# Autodesk Inventor assembly: servo_holder-asm
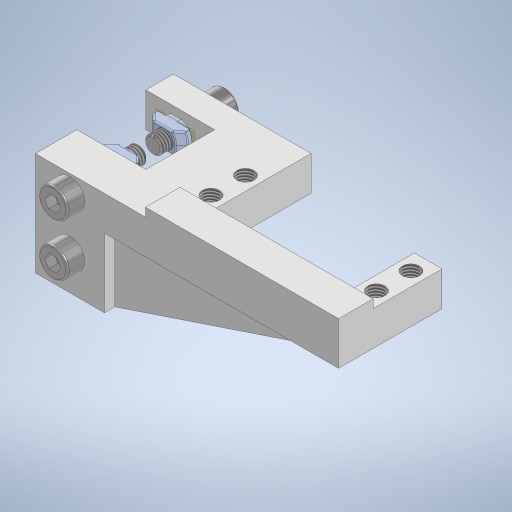
[picture p0: Inventor's stored thumbnail of the model, 512x512]
Saved by Autodesk Inventor 2024 (Build 280153000, 153)
## iProperties
Created: 2025-12-27
Part Number: servo_holder-asm
Document SubType Name: Assembly
Designer: schar
Author: schar
## Documents named in this file (5)
- C:\Users\schar\Desktop\projectBlueprint\AMSTS\hardware\servo_holder-asm.iam
- C:\Users\schar\Desktop\projectBlueprint\AMSTS\hardware\servo_holder.ipt
- C:\Users\schar\Desktop\projectBlueprint\AMSTS\hardware\tnut_m5_2020.ipt
- C:\Users\schar\Documents\Inventor\Content Center Files\R2024\en-US\ISO 4762(1)\DIN EN ISO 4762 - M5 x 20.ipt
- C:\Users\schar\Documents\Inventor\Content Center Files\R2024\en-US\ISO 4762(1)\DIN EN ISO 4762 - M5 x 16.ipt
## Components (7 placed, 4 different names)
1. servo_holder:1 — Rigid:3, Rigid:1, Rigid:2, Mate:1, Mate:2, Mate:3
2. tnut_m5_2020:1 — Rigid:2, Mate:4
3. tnut_m5_2020:2 — Rigid:1, Mate:6
4. tnut_m5_2020:3 — Rigid:3, Mate:5
5. DIN EN ISO 4762 M5 x 20:1 — Mate:1, Mate:6
6. DIN EN ISO 4762 M5 x 20:2 — Mate:2, Mate:5
7. DIN EN ISO 4762 M5 x 16:1 — Mate:3, Mate:4
## Relationships (9: Mate 6, WeldJoint 3)
- Rigid:3 [WeldJoint] (-0.159 mm): servo_holder:1 ↔ tnut_m5_2020:3
- Rigid:1 [WeldJoint] (-0.159 mm): servo_holder:1 ↔ tnut_m5_2020:2
- Rigid:2 [WeldJoint] (0.159 mm): servo_holder:1 ↔ tnut_m5_2020:1
- Mate:1: servo_holder:1 ↔ DIN EN ISO 4762 M5 x 20:1
- Mate:2: servo_holder:1 ↔ DIN EN ISO 4762 M5 x 20:2
- Mate:3: servo_holder:1 ↔ DIN EN ISO 4762 M5 x 16:1
- Mate:4: tnut_m5_2020:1 ↔ DIN EN ISO 4762 M5 x 16:1
- Mate:5: tnut_m5_2020:3 ↔ DIN EN ISO 4762 M5 x 20:2
- Mate:6: tnut_m5_2020:2 ↔ DIN EN ISO 4762 M5 x 20:1
